# Autodesk Inventor assembly: dsitributor
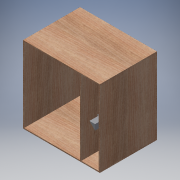
[picture p0: Inventor's stored thumbnail of the model, 180x180]
Saved by Autodesk Inventor 2018 (Build 220112000, 112)
## iProperties
Created: 2018-12-03
Part Number: dsitributor
Document SubType Name: Assembly
Designer: Bienvenue
Author: Bienvenue
## Documents named in this file (7)
- C:\Users\Bienvenue\Documents\Cours\PeiP2\Arduino\Projet\représentation3D\distributeur.iam
- C:\Users\Bienvenue\Documents\Cours\PeiP2\Arduino\Projet\représentation3D\planche_gauche.ipt
- C:\Users\Bienvenue\Documents\Cours\PeiP2\Arduino\Projet\représentation3D\planche derrière.ipt
- C:\Users\Bienvenue\Documents\Cours\PeiP2\Arduino\Projet\représentation3D\planche_bas.ipt
- C:\Users\Bienvenue\Documents\Cours\PeiP2\Arduino\Projet\représentation3D\cloison_porte-monnayeur.ipt
- C:\Users\Bienvenue\Documents\Cours\PeiP2\Arduino\Projet\représentation3D\monnayeur.ipt
- C:\Users\Bienvenue\Documents\Cours\PeiP2\Arduino\Projet\représentation3D\cale_monnayeur.ipt
## Components (8 placed, 6 different names)
1. planche_gauche:1 — Mate:1, Flush:1, Flush:3, Flush:6, Mate:4, Mate:7
2. planche_gauche:2 — Mate:2, Flush:2, Flush:4, Flush:5, Flush:11, Mate:10, Flush:13
3. planche derrière:1 — Mate:3, Flush:5, Flush:6, Mate:4, Flush:10
4. planche_bas:1 — Mate:1, Mate:2, Flush:1, Flush:2, Flush:3, Flush:4, Mate:3, Flush:12, Mate:9, Mate:12
5. planche_bas:2 — Mate:7, Flush:10, Flush:11, Mate:8
6. cloison_porte-monnayeur:1 — Mate:8, Flush:12, Mate:9
7. monnayeur:1 — Mate:11, Flush:14, Mate:13
8. cale_monnayeur:1 — Mate:10, Flush:13, Mate:11, Mate:12, Flush:14, Mate:13
## Relationships (22: Mate 11, Flush 11)
- Mate:1: planche_gauche:1 ↔ planche_bas:1
- Mate:2: planche_gauche:2 ↔ planche_bas:1
- Flush:1: planche_gauche:1 ↔ planche_bas:1
- Flush:2: planche_gauche:2 ↔ planche_bas:1
- Flush:3: planche_gauche:1 ↔ planche_bas:1
- Flush:4: planche_gauche:2 ↔ planche_bas:1
- Mate:3: planche derrière:1 ↔ planche_bas:1
- Flush:5: planche_gauche:2 ↔ planche derrière:1
- Flush:6: planche_gauche:1 ↔ planche derrière:1
- Mate:4: planche_gauche:1 ↔ planche derrière:1
- Mate:7: planche_gauche:1 ↔ planche_bas:2
- Flush:10: planche derrière:1 ↔ planche_bas:2
- Flush:11: planche_gauche:2 ↔ planche_bas:2
- Mate:8: planche_bas:2 ↔ cloison_porte-monnayeur:1
- Flush:12: planche_bas:1 ↔ cloison_porte-monnayeur:1
- Mate:9: planche_bas:1 ↔ cloison_porte-monnayeur:1
- Mate:10: planche_gauche:2 ↔ cale_monnayeur:1
- Flush:13: planche_gauche:2 ↔ cale_monnayeur:1
- Mate:11: monnayeur:1 ↔ cale_monnayeur:1
- Mate:12 (177.8 mm): planche_bas:1 ↔ cale_monnayeur:1
- Flush:14 (-50.8 mm): monnayeur:1 ↔ cale_monnayeur:1
- Mate:13: monnayeur:1 ↔ cale_monnayeur:1
